# Autodesk Inventor assembly: FlyingUGV
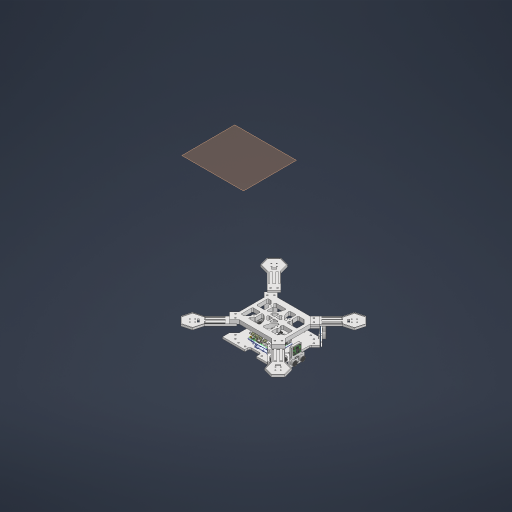
[picture p0: Inventor's stored thumbnail of the model, 512x512]
Saved by Autodesk Inventor 2023 (Build 270158000, 158)
## iProperties
Created: 2023-02-06
Part Number: FlyingUGV
Document SubType Name: Assembly
Designer: Michael
Author: Michael
## Documents named in this file (18)
- C:\Users\Michael\Documents\GitHub\SDP-Kepler-1708b\FlyingUGV.iam
- C:\Users\Michael\Documents\GitHub\SDP-Kepler-1708b\Arm.ipt
- C:\Users\Michael\Documents\GitHub\SDP-Kepler-1708b\Base.ipt
- Electronics Panel.ipt
- C:\Users\Michael\Documents\GitHub\SDP-Kepler-1708b\Camera Mount.ipt
- C:\Users\Michael\Documents\GitHub\SDP-Kepler-1708b\Top.ipt
- C:\Users\Michael\Documents\GitHub\SDP-Kepler-1708b\Electronics\ESC F45A\F45A.ipt
- C:\Users\Michael\Documents\GitHub\SDP-Kepler-1708b\Electronics\navio2\NAVIO2.ipt
- C:\Users\Michael\Documents\GitHub\SDP-Kepler-1708b\Electronics\navio2\hardware-master\VibroNavio2bot_rev_A.ipt
- C:\Users\Michael\Documents\GitHub\SDP-Kepler-1708b\Electronics\navio2\hardware-master\VibroNavio2top_rev_A.ipt
- C:\Users\Michael\Documents\GitHub\SDP-Kepler-1708b\Electronics\raspberry-pi-3-model-b\Solidworks Complete Assembly\Raspberry Pi 3.ipt
- C:\Users\Michael\Documents\GitHub\SDP-Kepler-1708b\Electronics\tattu-4s-6750mah-lipo-battery\Tattu_4S_6750mAh_25C\Tattu_4S_6750mAh_25C.ipt
- C:\Users\Michael\Documents\GitHub\SDP-Kepler-1708b\soporte.ipt
- C:\Users\Michael\Documents\GitHub\SDP-Kepler-1708b\Electronics\HC-SR04\HC-SR04-UltrasonicSensor v7.ipt
- C:\Users\Michael\Documents\GitHub\SDP-Kepler-1708b\Electronics\Raspberry pi 3 cam V2,1\Cam V2.1 v1.ipt
- C:\Users\Michael\Documents\GitHub\SDP-Kepler-1708b\Electronics\RP-lidar-A1\RP-lidar-A1.iam
- C:\Users\Michael\Documents\Motor Mounts.ipt
- C:\Users\Michael\Documents\GitHub\SDP-Kepler-1708b\STLs\Standoff.ipt
## Components (24 placed, 16 different names)
1. Arm:1 — Mate:62
2. Electronics Panel:1 — Mate:1, Mate:6, Mate:7, Mate:8, Mate:19, Mate:32, Flush:5, Flush:6, Mate:50, Mate:53, Mate:60, Mate:61, Flush:7
3. Camera Mount:1 — Mate:6, Mate:7, Mate:8, Mate:34, Flush:3, Flush:4, Mate:41, Mate:42
4. Top:1 — Mate:19, Mate:43, Mate:62
5. F45A:1 — Mate:11, Mate:51, Mate:52, Mate:53
6. F45A:2 — Mate:11, Mate:51, Mate:52
7. NAVIO2:1 — Mate:16, Flush:1, Flush:2
8. VibroNavio2bot_rev_A:1 — Mate:1, Mate:4, Mate:5
9. VibroNavio2top_rev_A:1 — Mate:4, Mate:5, Mate:13, Mate:14, Mate:15
10. Raspberry Pi 3:1 — Mate:13, Mate:14, Mate:15, Mate:16, Flush:1, Flush:2
11. Arm:2
12. Arm:3
13. Arm:4
14. Tattu_4S_6750mAh_25C:1 — Mate:32
15. HC-SR04-UltrasonicSensor v7:1 — Mate:39, Mate:40
16. Cam V2.1 v1:1 — Mate:34, Flush:3, Flush:4
17. RP-lidar-A1:1 [sub-assembly] — Mate:43
18. soporte:2 — Mate:39, Mate:40, Flush:5
19. HC-SR04-UltrasonicSensor v7:2 — Mate:41, Mate:42
20. soporte:3 — Flush:6, Mate:48, Mate:49
21. HC-SR04-UltrasonicSensor v7:3 — Mate:48, Mate:49
22. Motor Mounts:1 — Mate:50, Mate:60, Mate:61
23. Standoff:1
24. Standoff:2 — Flush:7
## Relationships (35: Mate 28, Flush 7)
- Mate:1: Electronics Panel:1 ↔ VibroNavio2bot_rev_A:1
- Mate:4: VibroNavio2bot_rev_A:1 ↔ VibroNavio2top_rev_A:1
- Mate:5: VibroNavio2bot_rev_A:1 ↔ VibroNavio2top_rev_A:1
- Mate:6: Electronics Panel:1 ↔ Camera Mount:1
- Mate:7: Electronics Panel:1 ↔ Camera Mount:1
- Mate:8: Electronics Panel:1 ↔ Camera Mount:1
- Mate:11 (12.7 mm): F45A:1 ↔ F45A:2
- Mate:13: VibroNavio2top_rev_A:1 ↔ Raspberry Pi 3:1
- Mate:14: VibroNavio2top_rev_A:1 ↔ Raspberry Pi 3:1
- Mate:15: VibroNavio2top_rev_A:1 ↔ Raspberry Pi 3:1
- Mate:16 (10.16 mm): NAVIO2:1 ↔ Raspberry Pi 3:1
- Flush:1: NAVIO2:1 ↔ Raspberry Pi 3:1
- Flush:2: NAVIO2:1 ↔ Raspberry Pi 3:1
- Mate:19 (47.625 mm): Electronics Panel:1 ↔ Top:1
- Mate:32: Electronics Panel:1 ↔ Tattu_4S_6750mAh_25C:1
- Mate:34: Camera Mount:1 ↔ Cam V2.1 v1:1
- Flush:3 (3.3782 mm): Camera Mount:1 ↔ Cam V2.1 v1:1
- Flush:4 (2.54 mm): Camera Mount:1 ↔ Cam V2.1 v1:1
- Mate:39: HC-SR04-UltrasonicSensor v7:1 ↔ soporte:2
- Mate:40: HC-SR04-UltrasonicSensor v7:1 ↔ soporte:2
- Mate:41: Camera Mount:1 ↔ HC-SR04-UltrasonicSensor v7:2
- Mate:42: Camera Mount:1 ↔ HC-SR04-UltrasonicSensor v7:2
- Mate:43: Top:1 ↔ RP-lidar-A1:1
- Flush:5: Electronics Panel:1 ↔ soporte:2
- Flush:6: Electronics Panel:1 ↔ soporte:3
- Mate:48: soporte:3 ↔ HC-SR04-UltrasonicSensor v7:3
- Mate:49: soporte:3 ↔ HC-SR04-UltrasonicSensor v7:3
- Mate:50: Electronics Panel:1 ↔ Motor Mounts:1
- Mate:51: F45A:1 ↔ F45A:2
- Mate:52: F45A:1 ↔ F45A:2
- Mate:53: Electronics Panel:1 ↔ F45A:1
- Mate:60: Electronics Panel:1 ↔ Motor Mounts:1
- Mate:61: Electronics Panel:1 ↔ Motor Mounts:1
- Mate:62: Arm:1 ↔ Top:1
- Flush:7: Electronics Panel:1 ↔ Standoff:2
